# Autodesk Inventor assembly: plug-craft
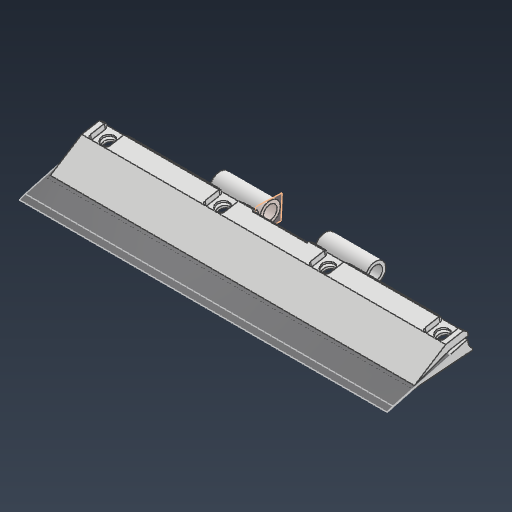
[picture p0: Inventor's stored thumbnail of the model, 512x512]
Saved by Autodesk Inventor 2023 (Build 270158000, 158)
## iProperties
Created: 2025-07-07
Part Number: plug-craft
Document SubType Name: Assembly
Designer: szymo
Author: szymo
## Documents named in this file (4)
- D:\tech\robotyka\robots\evangelion\inventor-project\plug-craft.iam
- D:\tech\robotyka\robots\evangelion\inventor-project\plog.ipt
- D:\tech\robotyka\robots\evangelion\inventor-project\plug-hold.ipt
- D:\tech\robotyka\robots\evangelion\inventor-project\plog-uphold.ipt
## Components (3 placed, 3 different names)
1. plog:1
2. plug-hold:1 — Flush:1, Flush:2
3. plog-uphold:1 — Flush:1, Flush:2
## Relationships (2: Flush 2)
- Flush:1: plug-hold:1 ↔ plog-uphold:1
- Flush:2: plug-hold:1 ↔ plog-uphold:1
